# Autodesk Inventor assembly: Assembly1
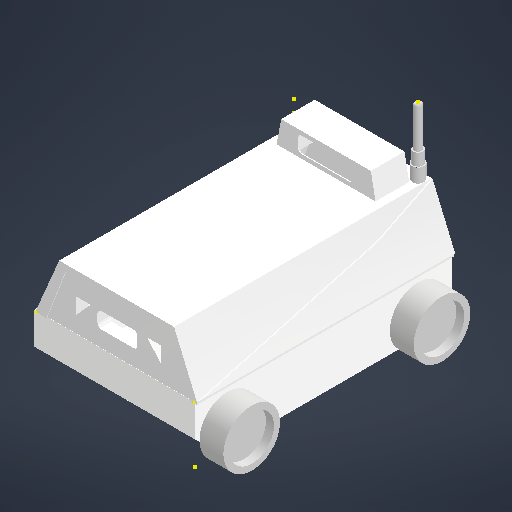
[picture p0: Inventor's stored thumbnail of the model, 512x512]
Saved by Autodesk Inventor 2027 (Build 310192060, 192F)
## iProperties
Created: 2026-06-05
Part Number: Assembly1
Document SubType Name: Assembly
Designer: CatKartikSUPREMEPC
Author: CatKartikSUPREMEPC
## Documents named in this file (5)
- C:\Users\CatKartikSUPREMEPC\Documents\Stasis Design\Assemblies\Assembly1.iam
- C:\Users\CatKartikSUPREMEPC\Documents\Stasis Design\Body.ipt
- C:\Users\CatKartikSUPREMEPC\Documents\Stasis Design\Cover.ipt
- C:\Users\CatKartikSUPREMEPC\Documents\Stasis Design\Antenna that serves no purpose other than to look cool.ipt
- C:\Users\CatKartikSUPREMEPC\Documents\Stasis Design\wheel.ipt
## Components (5 placed, 4 different names)
1. Body:1
2. Antenna that serves no purpose other than to look cool:1 — Rotational:1
3. Cover:1 — Rotational:1
4. wheel:1
5. wheel:2
## Relationships (1: RevoluteJoint 1)
- Rotational:1 [RevoluteJoint]: Antenna that serves no purpose other than to look cool:1 ↔ Cover:1
